# Autodesk Inventor assembly: Outer
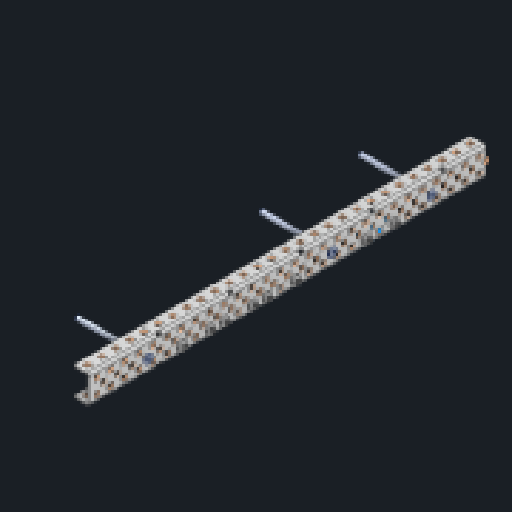
[picture p0: Inventor's stored thumbnail of the model, 512x512]
Saved by Autodesk Inventor 2025 (Build 290162000, 162)
## iProperties
Created: 2025-01-27
Part Number: Outer
Document SubType Name: Assembly
Designer: Averey Ku
Author: Averey Ku
## Documents named in this file (9)
- D:\VEX\High Stakes\CAD\V5\Chassis\Drivebay\Outer.iam
- D:\VEX\High Stakes\CAD\ROBOPROS-CAD-Inventor\Motion\Shaft LS\Bearing Flat Low Profile.ipt
- D:\VEX\High Stakes\CAD\ROBOPROS-CAD-Inventor\Structure\Hardware\Screw Nylon - Pan Head\NScrew Pan Head Threaded .500.ipt
- D:\VEX\High Stakes\CAD\ROBOPROS-CAD-Inventor\Structure\Hardware\Screw Steel - Star\SScrew Star Smooth 2.500.ipt
- D:\VEX\High Stakes\CAD\ROBOPROS-CAD-Inventor\Structure\Hardware\Screw Steel - Star.ipt
- D:\VEX\High Stakes\CAD\ROBOPROS-CAD-Inventor\Structure\Hardware\Nut Keps.ipt
- D:\VEX\High Stakes\CAD\ROBOPROS-CAD-Inventor\Structure\Hardware\Nut Nylon\Nut Nylon - White.ipt
- D:\VEX\High Stakes\CAD\ROBOPROS-CAD-Inventor\Structure\Hardware\Nut Nylon.ipt
- D:\VEX\High Stakes\CAD\ROBOPROS-CAD-Inventor\Structure\C Channel\Aluminum 1x2x1\Alu C 1x2x1x28.ipt
## Components (27 placed, 6 different names)
1. Bearing Flat Low Profile:1 — Insert:19, Insert:20, Insert:28
2. Bearing Flat Low Profile:2 — Insert:21, Insert:22, Insert:32, Mate:3
3. Bearing Flat Low Profile:3 — Insert:23, Insert:24, Insert:44
4. NScrew Pan Head Threaded .500:1 — Insert:33
5. NScrew Pan Head Threaded .500:2 — Insert:35
6. NScrew Pan Head Threaded .500:3 — Insert:37
7. NScrew Pan Head Threaded .500:4 — Insert:36
8. NScrew Pan Head Threaded .500:5 — Insert:39, Mate:4
9. NScrew Pan Head Threaded .500:6 — Insert:38
10. SScrew Star Smooth 2.500:1 — Insert:27
11. SScrew Star Smooth 2.500:3 — Insert:26
12. SScrew Star Smooth 2.500:4 — Insert:25
13. Nut Keps:2 — Insert:43
14. Nut Keps:3 — Insert:41
15. Nut Keps:4 — Insert:42
16. Nut Nylon - White:1 — Insert:19
17. Nut Nylon - White:2 — Insert:21
18. Nut Nylon - White:3 — Insert:20, Mate:1
19. Nut Nylon - White:4 — Insert:22
20. Nut Nylon - White:5 — Insert:23, Mate:4
21. Nut Nylon - White:6 — Insert:24
22. Alu C 1x2x1x28:1 — Flush:1, Flush:2, Flush:3, Insert:25, Insert:26, Insert:27, Insert:28, Mate:1, Insert:31, Mate:2, Insert:32, Mate:3, Insert:33, Insert:34, Insert:35, Insert:36, Insert:37, Insert:38, Insert:39, Insert:40, Insert:41, Insert:42, Insert:43, Insert:44
23. Bearing Flat Low Profile:4 — Insert:31, Mate:2
24. Nut Nylon - White:7
25. Nut Nylon - White:8
26. NScrew Pan Head Threaded .500:7 — Insert:34
27. NScrew Pan Head Threaded .500:8 — Insert:40
## Relationships (33: Insert 26, Mate 4, Flush 3)
- Insert:19 (1.27 mm): Bearing Flat Low Profile:1 ↔ Nut Nylon - White:1
- Insert:20 (1.27 mm): Bearing Flat Low Profile:1 ↔ Nut Nylon - White:3
- Insert:21 (1.27 mm): Bearing Flat Low Profile:2 ↔ Nut Nylon - White:2
- Insert:22 (1.27 mm): Bearing Flat Low Profile:2 ↔ Nut Nylon - White:4
- Insert:23 (1.27 mm): Bearing Flat Low Profile:3 ↔ Nut Nylon - White:5
- Insert:24 (1.27 mm): Bearing Flat Low Profile:3 ↔ Nut Nylon - White:6
- Flush:1 (-177.8 mm): Alu C 1x2x1x28:1
- Flush:2 (-12.7 mm): Alu C 1x2x1x28:1
- Flush:3: Alu C 1x2x1x28:1
- Insert:25 (1.5875 mm): SScrew Star Smooth 2.500:4 ↔ Alu C 1x2x1x28:1
- Insert:26 (1.5875 mm): SScrew Star Smooth 2.500:3 ↔ Alu C 1x2x1x28:1
- Insert:27 (1.5875 mm): SScrew Star Smooth 2.500:1 ↔ Alu C 1x2x1x28:1
- Insert:28: Bearing Flat Low Profile:1 ↔ Alu C 1x2x1x28:1
- Mate:1: Nut Nylon - White:3 ↔ Alu C 1x2x1x28:1
- [Insert] (1.27 mm): Bearing Flat Low Profile:4 ↔ Nut Nylon - White:7
- [Insert] (1.27 mm): Bearing Flat Low Profile:4 ↔ Nut Nylon - White:8
- Insert:31: Alu C 1x2x1x28:1 ↔ Bearing Flat Low Profile:4
- Mate:2: Alu C 1x2x1x28:1 ↔ Bearing Flat Low Profile:4
- Insert:32: Bearing Flat Low Profile:2 ↔ Alu C 1x2x1x28:1
- Mate:3: Bearing Flat Low Profile:2 ↔ Alu C 1x2x1x28:1
- Insert:33: NScrew Pan Head Threaded .500:1 ↔ Alu C 1x2x1x28:1
- Insert:34: Alu C 1x2x1x28:1 ↔ NScrew Pan Head Threaded .500:7
- Insert:35: NScrew Pan Head Threaded .500:2 ↔ Alu C 1x2x1x28:1
- Insert:36: NScrew Pan Head Threaded .500:4 ↔ Alu C 1x2x1x28:1
- Insert:37: NScrew Pan Head Threaded .500:3 ↔ Alu C 1x2x1x28:1
- Insert:38: NScrew Pan Head Threaded .500:6 ↔ Alu C 1x2x1x28:1
- Insert:39: NScrew Pan Head Threaded .500:5 ↔ Alu C 1x2x1x28:1
- Insert:40: Alu C 1x2x1x28:1 ↔ NScrew Pan Head Threaded .500:8
- Insert:41: Nut Keps:3 ↔ Alu C 1x2x1x28:1
- Insert:42: Nut Keps:4 ↔ Alu C 1x2x1x28:1
- Insert:43: Nut Keps:2 ↔ Alu C 1x2x1x28:1
- Insert:44: Bearing Flat Low Profile:3 ↔ Alu C 1x2x1x28:1
- Mate:4: NScrew Pan Head Threaded .500:5 ↔ Nut Nylon - White:5
## Named parameters: d74_d57 = 1.27 mm, d75_d58 = 1.27 mm
